# Autodesk Inventor assembly: Assembly_Cube_Z_Stage_Objective_Holder_XY_Stage
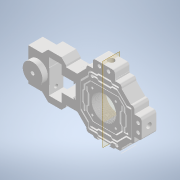
[picture p0: Inventor's stored thumbnail of the model, 180x180]
Saved by Autodesk Inventor 2022.3 (Build 263350000, 350)
## iProperties
Created: 2022-07-14
Part Number: Assembly_Cube_Z_Stage_Objective_Holder_XY_Stage
Document SubType Name: Assembly
Designer: bingoeleda
Author: bingoeleda
## Documents named in this file (3)
- G:\My Drive\ASP - M.Sc. Photonics\Practical Modules\MODULE 4 - Master Thesis\2.Experiments\Modules\9.Adjustable_Z_Stage_Module\Manually_driven_Tilted__MGN12H_XZ_Stage\Assembly_Cube_Z_Stage_Objective_XY_Stage.iam
- G:\My Drive\ASP - M.Sc. Photonics\Practical Modules\MODULE 4 - Master Thesis\2.Experiments\Modules\9.Adjustable_Z_Stage_Module\Manually_driven_Tilted__MGN12H_XZ_Stage\20_Cube_Inser_Flexuremanipulator_m3_screws_v3.ipt
- G:\My Drive\ASP - M.Sc. Photonics\Practical Modules\MODULE 4 - Master Thesis\2.Experiments\Modules\9.Adjustable_Z_Stage_Module\Manually_driven_Tilted__MGN12H_XZ_Stage\30_Cube_Cube_Z_Focus_XY_Stage_MGN_NEMA_belt_pushing_slide_v3.ipt
## Components (2 placed, 2 different names)
1. 20_Cube_Inser_Flexuremanipulator_m3_screws_v3:1 — Mate:1, Mate:2, Flush:1, Mate:4, Mate:5, Mate:6, Mate:7
2. 30_Cube_Cube_Z_Focus_XY_Stage_MGN_NEMA_belt_pushing_slide_v3:1 — Mate:1, Mate:2, Flush:1, Mate:4
## Relationships (7: Mate 6, Flush 1)
- Mate:1: 20_Cube_Inser_Flexuremanipulator_m3_screws_v3:1 ↔ 30_Cube_Cube_Z_Focus_XY_Stage_MGN_NEMA_belt_pushing_slide_v3:1
- Mate:2: 20_Cube_Inser_Flexuremanipulator_m3_screws_v3:1 ↔ 30_Cube_Cube_Z_Focus_XY_Stage_MGN_NEMA_belt_pushing_slide_v3:1
- Flush:1: 20_Cube_Inser_Flexuremanipulator_m3_screws_v3:1 ↔ 30_Cube_Cube_Z_Focus_XY_Stage_MGN_NEMA_belt_pushing_slide_v3:1
- Mate:4: 20_Cube_Inser_Flexuremanipulator_m3_screws_v3:1 ↔ 30_Cube_Cube_Z_Focus_XY_Stage_MGN_NEMA_belt_pushing_slide_v3:1
- Mate:5: 20_Cube_Inser_Flexuremanipulator_m3_screws_v3:1
- Mate:6: 20_Cube_Inser_Flexuremanipulator_m3_screws_v3:1
- Mate:7: 20_Cube_Inser_Flexuremanipulator_m3_screws_v3:1
